# Autodesk Inventor assembly: SanladererBowdenExtruder
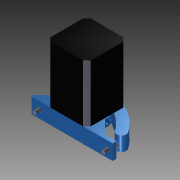
[picture p0: Inventor's stored thumbnail of the model, 180x180]
Saved by Autodesk Inventor 2015 SP1 (Build 190203100, 203)
## iProperties
Created: 2015-01-11
Part Number: SanladererBowdenExtruder
Document SubType Name: Assembly
Designer: Jack
Mass: 146.826 g
Surface Area: 300.593 cm^2
Volume: 138.026 cm^3
Density: 1.06375 g/cm^3
Author: Jack
Title: Sanladerer Bowden Extruder
## Documents named in this file (9)
- C:\Users\Jack\ownCloud\Projects\CrossBot\InventorModel\Extruder\SanladererBowdenExtruder\SanladererBowdenExtruder.iam
- C:\Users\Jack\ownCloud\Projects\CrossBot\InventorModel\Extruder\SanladererBowdenExtruder\SanladererBowdenArm.ipt
- C:\Users\Jack\ownCloud\Projects\CrossBot\InventorModel\Extruder\SanladererBowdenExtruder\SanladererBowdenBody.ipt
- C:\Users\Jack\ownCloud\Projects\CrossBot\InventorModel\Electronics\Motors\StepperMotorNema17x60mm.ipt
- C:\Users\Jack\ownCloud\Projects\CrossBot\InventorModel\Hardware\Extruder\DriveGearMK8.ipt
- C:\Users\Jack\ownCloud\Projects\CrossBot\InventorModel\Hardware\Bearing\BearingRadialBall\BearingRadialBall624zz.ipt
- C:\Users\Jack\ownCloud\Projects\CrossBot\InventorModel\Hardware\BoltWashers\BoltWasher3\BoltWasher3x18.iam
- C:\Users\Jack\ownCloud\Projects\CrossBot\InventorModel\Hardware\BoltWashers\BoltWasher4\BoltWasher4x18.iam
- C:\Users\Jack\ownCloud\Projects\CrossBot\InventorModel\Hardware\BoltWashers\BoltWasher4\BoltWasher4x10.iam
## Components (12 placed, 8 different names)
1. SanladererBowdenArm:1 — Mate:8, Mate:12, Mate:13, Mate:14, Mate:46, Mate:47, Mate:51, Mate:52
2. SanladererBowdenBody:1 — Mate:5, Mate:6, Mate:7, Mate:43, Mate:44, Mate:45, Mate:48, Mate:49, Mate:50, Mate:53, Mate:54, Mate:55, Mate:56
3. StepperMotorNema17x60mm:1 — Mate:5, Mate:6, Mate:7, Mate:8, Mate:10, Mate:11, Mate:12
4. DriveGearMK8:1 — Mate:10, Mate:11
5. BoltWasher3x18:1 [sub-assembly] — Mate:45, Mate:49
6. BoltWasher3x18:2 [sub-assembly] — Mate:44, Mate:48
7. BoltWasher3x18:3 [sub-assembly] — Mate:43, Mate:50
8. BoltWasher3x18:4 [sub-assembly] — Mate:46, Mate:47
9. BoltWasher4x18:1 [sub-assembly] — Mate:51, Mate:52
10. BearingRadialBall624zz:1 — Mate:13, Mate:14
11. BoltWasher4x10:1 [sub-assembly] — Mate:53, Mate:56
12. BoltWasher4x10:2 [sub-assembly] — Mate:54, Mate:55
## Relationships (23: Mate 23)
- Mate:5: SanladererBowdenBody:1 ↔ StepperMotorNema17x60mm:1
- Mate:6: SanladererBowdenBody:1 ↔ StepperMotorNema17x60mm:1
- Mate:7: SanladererBowdenBody:1 ↔ StepperMotorNema17x60mm:1
- Mate:8: SanladererBowdenArm:1 ↔ StepperMotorNema17x60mm:1
- Mate:10: StepperMotorNema17x60mm:1 ↔ DriveGearMK8:1
- Mate:11 (3 mm): StepperMotorNema17x60mm:1 ↔ DriveGearMK8:1
- Mate:12: SanladererBowdenArm:1 ↔ StepperMotorNema17x60mm:1
- Mate:13: SanladererBowdenArm:1 ↔ BearingRadialBall624zz:1
- Mate:14: SanladererBowdenArm:1 ↔ BearingRadialBall624zz:1
- Mate:43: SanladererBowdenBody:1 ↔ BoltWasher3x18:3
- Mate:44: SanladererBowdenBody:1 ↔ BoltWasher3x18:2
- Mate:45: SanladererBowdenBody:1 ↔ BoltWasher3x18:1
- Mate:46: SanladererBowdenArm:1 ↔ BoltWasher3x18:4
- Mate:47: SanladererBowdenArm:1 ↔ BoltWasher3x18:4
- Mate:48: SanladererBowdenBody:1 ↔ BoltWasher3x18:2
- Mate:49: SanladererBowdenBody:1 ↔ BoltWasher3x18:1
- Mate:50: SanladererBowdenBody:1 ↔ BoltWasher3x18:3
- Mate:51: SanladererBowdenArm:1 ↔ BoltWasher4x18:1
- Mate:52: SanladererBowdenArm:1 ↔ BoltWasher4x18:1
- Mate:53: SanladererBowdenBody:1 ↔ BoltWasher4x10:1
- Mate:54: SanladererBowdenBody:1 ↔ BoltWasher4x10:2
- Mate:55: SanladererBowdenBody:1 ↔ BoltWasher4x10:2
- Mate:56: SanladererBowdenBody:1 ↔ BoltWasher4x10:1
